# Autodesk Inventor assembly: Adamant Cover
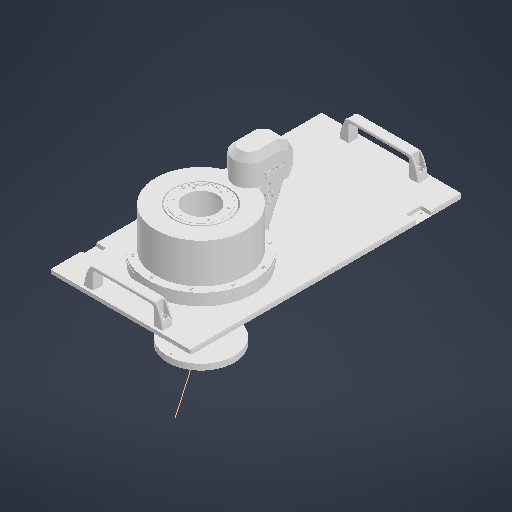
[picture p0: Inventor's stored thumbnail of the model, 512x512]
Saved by Autodesk Inventor 2026.2 (Build 302298000, 298)
## iProperties
Created: 2026-01-05
Part Number: Adamant Cover
Document SubType Name: Assembly
Designer: mumin
Author: mumin
## Documents named in this file (12)
- C:\GitHub\In-situ-monitoring-of-powder-bed-fusion-additive-manufacturing\system_development\Adamant\v0.2\hardware_development\Cover parts\Adamant Cover.iam
- C:\GitHub\In-situ-monitoring-of-powder-bed-fusion-additive-manufacturing\system_development\Adamant\v0.2\hardware_development\Cover parts\New Thermal Housing.ipt
- C:\GitHub\In-situ-monitoring-of-powder-bed-fusion-additive-manufacturing\system_development\Adamant\v0.2\hardware_development\Cover parts\New Thermal Lid.ipt
- C:\GitHub\In-situ-monitoring-of-powder-bed-fusion-additive-manufacturing\system_development\Adamant\v0.2\hardware_development\Cover parts\SealedGlassRing.ipt
- C:\GitHub\In-situ-monitoring-of-powder-bed-fusion-additive-manufacturing\system_development\Adamant\v0.2\hardware_development\Cover parts\Thermal Chamber Cover.ipt
- C:\GitHub\In-situ-monitoring-of-powder-bed-fusion-additive-manufacturing\system_development\Adamant\v0.2\hardware_development\Cover parts\Handle.ipt
- C:\GitHub\In-situ-monitoring-of-powder-bed-fusion-additive-manufacturing\system_development\Adamant\v0.2\hardware_development\Cover parts\Horse Shoe .ipt
- C:\GitHub\In-situ-monitoring-of-powder-bed-fusion-additive-manufacturing\system_development\Adamant\v0.2\hardware_development\Cover parts\Thermal Cylinder Segments\C .Replace - 10.ipt
- C:\GitHub\In-situ-monitoring-of-powder-bed-fusion-additive-manufacturing\system_development\Adamant\v0.2\hardware_development\Cover parts\Thermal Cylinder Segments.ipt
- C:\GitHub\In-situ-monitoring-of-powder-bed-fusion-additive-manufacturing\system_development\Adamant\v0.2\hardware_development\Cover parts\Thermal Cylinder Segments\C .Replace - Face.ipt
- C:\GitHub\In-situ-monitoring-of-powder-bed-fusion-additive-manufacturing\system_development\Adamant\v0.2\hardware_development\Cover parts\Xi-410-Camera-with-29°-x-18°-Lens\Xi 410 Camera with 29° x.iam
- C:\GitHub\In-situ-monitoring-of-powder-bed-fusion-additive-manufacturing\system_development\Adamant\v0.2\hardware_development\Cover parts\substrate plate.ipt
## Components (11 placed, 10 different names)
1. New Thermal Housing:1 — Mate:1, Mate:2, Mate:3, Insert:1, Insert:2, Insert:7, Insert:8, Insert:9, Insert:11
2. New Thermal Lid:1 — Mate:1, Mate:2, Mate:3
3. SealedGlassRing:1 — Insert:1, Insert:2, Insert:3, Insert:4
4. Thermal Chamber Cover:1 — Insert:3, Insert:4, Insert:5, Insert:6, Insert:12
5. Handle:1 — Insert:5
6. Handle:2 — Insert:6
7. Horse Shoe :1 — Insert:7, Insert:8
8. C .Replace - 10:1 — Insert:9, Insert:10
9. C .Replace - Face:2 — Insert:10
10. Xi 410 Camera with 29° x:1 [sub-assembly] — Insert:11
11. substrate plate:1 — Insert:12
## Relationships (15: Insert 12, Mate 3)
- Mate:1: New Thermal Housing:1 ↔ New Thermal Lid:1
- Mate:2: New Thermal Housing:1 ↔ New Thermal Lid:1
- Mate:3: New Thermal Housing:1 ↔ New Thermal Lid:1
- Insert:1: New Thermal Housing:1 ↔ SealedGlassRing:1
- Insert:2: New Thermal Housing:1 ↔ SealedGlassRing:1
- Insert:3: SealedGlassRing:1 ↔ Thermal Chamber Cover:1
- Insert:4: SealedGlassRing:1 ↔ Thermal Chamber Cover:1
- Insert:5: Thermal Chamber Cover:1 ↔ Handle:1
- Insert:6: Thermal Chamber Cover:1 ↔ Handle:2
- Insert:7: New Thermal Housing:1 ↔ Horse Shoe :1
- Insert:8: New Thermal Housing:1 ↔ Horse Shoe :1
- Insert:9: New Thermal Housing:1 ↔ C .Replace - 10:1
- Insert:10: C .Replace - 10:1 ↔ C .Replace - Face:2
- Insert:11: New Thermal Housing:1 ↔ Xi 410 Camera with 29° x:1
- Insert:12 (150 mm): Thermal Chamber Cover:1 ↔ substrate plate:1
